# Autodesk Inventor assembly: __VK_Hubeinehit_100
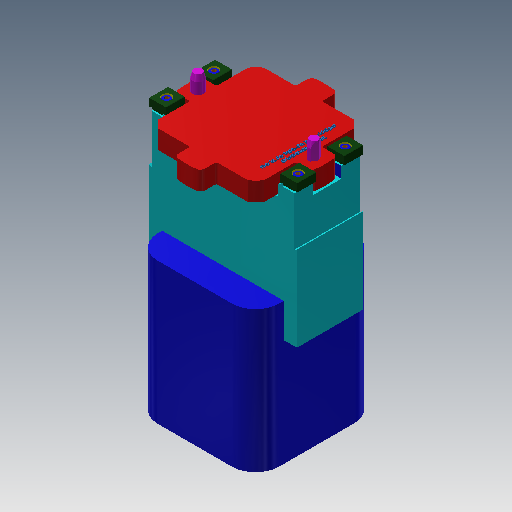
[picture p0: Inventor's stored thumbnail of the model, 512x512]
Saved by Autodesk Inventor 2019 (Build 230136000, 136)
## iProperties
Created: 2023-11-18
Part Number: __VK_Hubeinehit_100
Material: Generisch
Document SubType Name: Assembly
Designer: RP
Author: RP
## Documents named in this file (3)
- C:\Users\RP\Documents\Inventor\Projekt_Angelspule\_Verkettung\__VK_Hub-Dreheinheit.iam
- C:\Users\RP\Documents\Inventor\Projekt_Angelspule\_Verkettung\__VK_Hub-Dreheinheit_Basis.ipt
- C:\Users\RP\Documents\Inventor\Projekt_Angelspule\_Verkettung\__VK_Hub_Dreh_Einheit_Plattform.ipt
## Components (2 placed, 2 different names)
1. __VK_Hub-Dreheinheit_Basis:1 — Passend:1, Winkel:1, Passend:2, Fluchtend:2, Passend:3, Fluchtend:3
2. __VK_Hub_Dreh_Einheit_Plattform:1 — Passend:1, Winkel:1, Passend:2
## Relationships (6: Mate 3, Flush 2, Angle 1)
- Passend:1 [Mate]: __VK_Hub-Dreheinheit_Basis:1 ↔ __VK_Hub_Dreh_Einheit_Plattform:1
- Winkel:1 [Angle] (0 deg): __VK_Hub-Dreheinheit_Basis:1 ↔ __VK_Hub_Dreh_Einheit_Plattform:1
- Passend:2 [Mate]: __VK_Hub-Dreheinheit_Basis:1 ↔ __VK_Hub_Dreh_Einheit_Plattform:1
- Fluchtend:2 [Flush]: __VK_Hub-Dreheinheit_Basis:1
- Passend:3 [Mate]: __VK_Hub-Dreheinheit_Basis:1
- Fluchtend:3 [Flush] (41.02 mm): __VK_Hub-Dreheinheit_Basis:1
